# Autodesk Inventor assembly: belt_tender_1
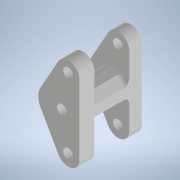
[picture p0: Inventor's stored thumbnail of the model, 180x180]
Saved by Autodesk Inventor 2020 (Build 240168000, 168)
## iProperties
Created: 2019-09-03
Part Number: belt_tender_1
Document SubType Name: Assembly
Designer: psrob
Author: psrob
## Documents named in this file (3)
- E:\projects-2\project dog gen2\hardware\belt_tender_1.iam
- E:\projects-2\project dog gen2\hardware\belt_tendor_1.ipt
- E:\projects-2\project dog gen2\hardware\belt_tender_2.ipt
## Components (2 placed, 2 different names)
1. belt_tendor_1:1 — Flush:1
2. belt_tender_2:1 — Flush:1
## Relationships (1: Flush 1)
- Flush:1: belt_tendor_1:1 ↔ belt_tender_2:1
